# Autodesk Inventor assembly: leg_connector_arm
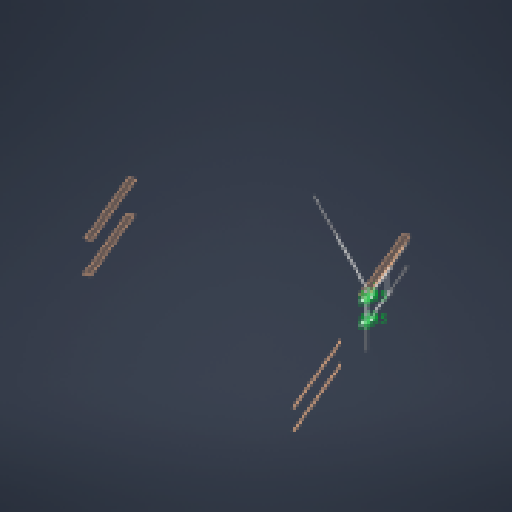
[picture p0: Inventor's stored thumbnail of the model, 512x512]
Saved by Autodesk Inventor 2023 (Build 270158000, 158)
## iProperties
Created: 2022-05-01
Part Number: leg_connector_arm
Document SubType Name: Assembly
Designer: Norbert Ligas
Mass: 651.448 g
Surface Area: 1185.23 cm^2
Volume: 116.903 cm^3
Density: 5.57254 g/cm^3
Author: Norbert Ligas
## Documents named in this file (4)
- C:\Users\norbe\Repozytoria\NormalMapScanner\stand_construction\parts\leg_connector_arm.iam
- C:\Users\norbe\Repozytoria\NormalMapScanner\stand_construction\parts\adjustable_arm.iam
- C:\Users\norbe\Repozytoria\NormalMapScanner\stand_construction\parts\adjustable_double_connector.iam
- C:\Users\norbe\Repozytoria\NormalMapScanner\stand_construction\parts\adjustable_leg.iam
## Components (3 placed, 3 different names)
1. adjustable_arm:1 [sub-assembly] — Mate:1, Mate:2
2. adjustable_leg:1 [sub-assembly] — Mate:1, Mate:2, Flush:2, Mate:5, Mate:6, Mate:7, Mate:8, Mate:9, Tangent:1
3. adjustable_double_connector:1 [sub-assembly] — Mate:7, Mate:8, Mate:9, Tangent:1
## Relationships (9: Mate 7, Flush 1, Tangent 1)
- Mate:1: adjustable_arm:1 ↔ adjustable_leg:1
- Mate:2: adjustable_arm:1 ↔ adjustable_leg:1
- Flush:2: adjustable_leg:1
- Mate:5: adjustable_leg:1
- Mate:6: adjustable_leg:1
- Mate:7: adjustable_leg:1 ↔ adjustable_double_connector:1
- Mate:8: adjustable_leg:1 ↔ adjustable_double_connector:1
- Mate:9: adjustable_leg:1 ↔ adjustable_double_connector:1
- Tangent:1: adjustable_leg:1 ↔ adjustable_double_connector:1
